# Autodesk Inventor assembly: BoxAssembly
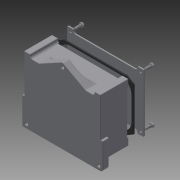
[picture p0: Inventor's stored thumbnail of the model, 180x180]
Saved by Autodesk Inventor 2014 SP2 (Build 180246200, 246)
## iProperties
Created: 2015-09-16
Part Number: BoxAssembly
Document SubType Name: Assembly
Designer: Lukasz Szmit
Author: Lukasz Szmit
## Documents named in this file (5)
- H:\Documents\Projects\mb\Ignition Module\Case\BoxAssembly.iam
- H:\Documents\Projects\mb\Ignition Module\Case\BoxOutline.ipt
- H:\Documents\Projects\mb\Ignition Module\Case\RubberLidSeal.ipt
- H:\Documents\Projects\mb\Ignition Module\Case\BoxLid.ipt
- H:\Documents\Projects\mb\Ignition Module\Case\M4x0.75_Bolt.ipt
## Components (7 placed, 4 different names)
1. ModuleBox:1 — Mate:1, Mate:2, Flush:1, Flush:2, Mate:3, Flush:3
2. RubberLidSeal:1 — Mate:1, Mate:2, Flush:1
3. BoxLid:1 — Flush:2, Mate:3, Flush:3, Insert:1, Insert:2, Insert:3, Insert:4
4. M4x0.75_Bolt:1 — Insert:1
5. M4x0.75_Bolt:2 — Insert:2
6. M4x0.75_Bolt:3 — Insert:3
7. M4x0.75_Bolt:4 — Insert:4
## Relationships (10: Insert 4, Mate 3, Flush 3)
- Mate:1 (10 mm): ModuleBox:1 ↔ RubberLidSeal:1
- Mate:2: ModuleBox:1 ↔ RubberLidSeal:1
- Flush:1: ModuleBox:1 ↔ RubberLidSeal:1
- Flush:2: ModuleBox:1 ↔ BoxLid:1
- Mate:3 (25 mm): ModuleBox:1 ↔ BoxLid:1
- Flush:3: ModuleBox:1 ↔ BoxLid:1
- Insert:1 (5 mm): BoxLid:1 ↔ M4x0.75_Bolt:1
- Insert:2 (5 mm): BoxLid:1 ↔ M4x0.75_Bolt:2
- Insert:3 (5 mm): BoxLid:1 ↔ M4x0.75_Bolt:3
- Insert:4 (5 mm): BoxLid:1 ↔ M4x0.75_Bolt:4
